# Autodesk Inventor assembly: Assembly1
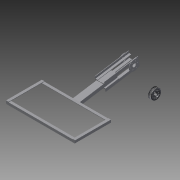
[picture p0: Inventor's stored thumbnail of the model, 180x180]
Saved by Autodesk Inventor 2015 (Build 190159000, 159)
## iProperties
Created: 2016-02-06
Part Number: Assembly1
Document SubType Name: Assembly
Designer: sethbattis
Author: sethbattis
## Documents named in this file (4)
- \\area51\team3566\cad\FRC 2016\Assembly1.iam
- \\area51\team3566\cad\FRC 2016\Prow rev2.ipt
- \\area51\team3566\cad\FRC 2016\Imported Components\42 tooth HTD Pulley half 2014.ipt\42 tooth HTD Pulley half 2014.ipt.ipt
- 42 tooth HTD Pulley half 2014.ipt
## Components (3 placed, 2 different names)
1. Prow rev2:1
2. 42 tooth HTD Pulley half 2014.ipt:1 — Mate:1, Mate:2, Mate:3
3. 42 tooth HTD Pulley half 2014.ipt:2 — Mate:1, Mate:2, Mate:3
## Relationships (3: Mate 3)
- Mate:1: 42 tooth HTD Pulley half 2014.ipt:1 ↔ 42 tooth HTD Pulley half 2014.ipt:2
- Mate:2: 42 tooth HTD Pulley half 2014.ipt:1 ↔ 42 tooth HTD Pulley half 2014.ipt:2
- Mate:3: 42 tooth HTD Pulley half 2014.ipt:1 ↔ 42 tooth HTD Pulley half 2014.ipt:2
